# Autodesk Inventor assembly: E006-Carter
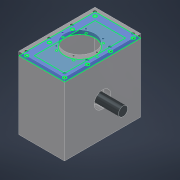
[picture p0: Inventor's stored thumbnail of the model, 180x180]
Saved by Autodesk Inventor 2021.3 (Build 253353000, 353)
## iProperties
Created: 2022-04-01
Part Number: E006-Carter
Document SubType Name: Assembly
Designer: remi
Author: remi
## Documents named in this file (4)
- C:\Users\remi\OneDrive\Documents\Cours\05-HEVS\S2fb\mechanic\CCo\project\Compressor\E006-Carter.iam
- C:\Users\remi\OneDrive\Documents\Cours\05-HEVS\S2fb\mechanic\CCo\project\Compressor\P016-Carter_corps.ipt
- C:\Users\remi\OneDrive\Documents\Cours\05-HEVS\S2fb\mechanic\CCo\project\Compressor\P015-Vilbrequin.ipt
- C:\Users\remi\OneDrive\Documents\Cours\05-HEVS\S2fb\mechanic\CCo\project\Compressor\P017-Carter_chapeau.ipt
## Components (3 placed, 3 different names)
1. P016-Carter_corps:1 — Mate:2, Flush:1, Flush:2, Mate:3
2. P015-Vilbrequin:1 — Mate:3
3. P017-Carter_chapeau:1 — Mate:2, Flush:1, Flush:2
## Relationships (4: Mate 2, Flush 2)
- Mate:2: P016-Carter_corps:1 ↔ P017-Carter_chapeau:1
- Flush:1: P016-Carter_corps:1 ↔ P017-Carter_chapeau:1
- Flush:2: P016-Carter_corps:1 ↔ P017-Carter_chapeau:1
- Mate:3: P016-Carter_corps:1 ↔ P015-Vilbrequin:1
